# Autodesk Inventor assembly: ASY Disk Micro filter v2.0
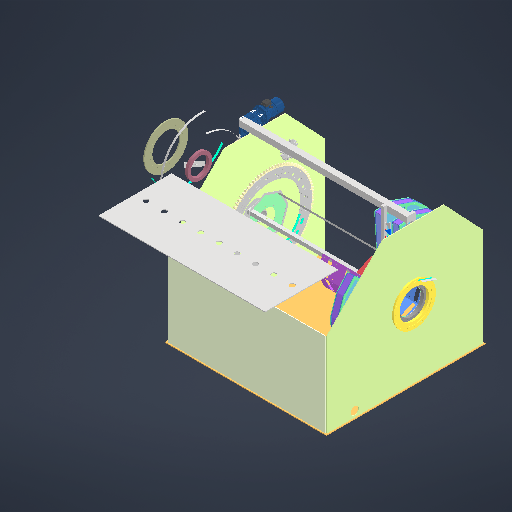
[picture p0: Inventor's stored thumbnail of the model, 512x512]
Saved by Autodesk Inventor 2026.2 (Build 302298010, 298A)
## iProperties
Created: 2023-08-31
Part Number: ASY Disk Micro filter v2.0
Document SubType Name: Assembly
Designer: admin
Stock Number: Дисковый_Фильтр
Author: admin
## Documents named in this file (38)
- C:\Users\admin\Documents\Inventor\DMF-Disk-Micro-Filter\ASY 000 ДМФ Disk Micro filter v2.0.iam
- C:\Users\admin\Documents\Inventor\DMF-Disk-Micro-Filter\Left wall v2.0.ipt
- C:\Users\admin\Documents\Inventor\DMF-Disk-Micro-Filter\Wall right v2.0.ipt
- C:\Users\admin\Documents\Inventor\DMF-Disk-Micro-Filter\DF1.03 Wall bottom v2.0.ipt
- C:\Users\admin\Documents\Inventor\DMF-Disk-Micro-Filter\DF1.04 Wall face v2.0.ipt
- C:\Users\admin\Documents\Inventor\DMF-Disk-Micro-Filter\ДМФ 021 кольцо прижимное нос v2.0.ipt
- C:\Users\admin\Documents\Inventor\DMF-Disk-Micro-Filter\ДМФ 000 размеры v2.0.ipt
- C:\Users\admin\Documents\Inventor\DMF-Disk-Micro-Filter\ДМФ 032 крышка Нос v2.0.ipt
- C:\Users\admin\Documents\Inventor\DMF-Disk-Micro-Filter\ДМФ 091 Постель НОС v2.0.ipt
- C:\Users\admin\Documents\Inventor\DMF-Disk-Micro-Filter\ДМФ 022 кольцо прижимное корма v2.0.ipt
- C:\Users\admin\Documents\Inventor\DMF-Disk-Micro-Filter\ДМФ 093 Постель КОРМА v2.0.ipt
- C:\Users\admin\Documents\Inventor\DMF-Disk-Micro-Filter\ДМФ 092 Коромысло КОРМА v2.0.ipt
- C:\Users\admin\Documents\Inventor\DMF-Disk-Micro-Filter\ДМФ 055 труба илоотвода v2.0.ipt
- C:\Users\admin\Documents\Inventor\DMF-Disk-Micro-Filter\ДМФ 033 держатель лотка v2.0.ipt
- C:\Users\admin\Documents\Inventor\DMF-Disk-Micro-Filter\ASY ДМФ лоток 050 илоотвод v2.0.iam
- C:\Users\admin\Documents\Inventor\DMF-Disk-Micro-Filter\ДМФ 092 Коромысло НОС v2.0.ipt
- C:\Users\admin\Documents\Inventor\DMF-Disk-Micro-Filter\ДМФ 066 Гребенка v2.0.ipt
- C:\Users\admin\Documents\Inventor\DMF-Disk-Micro-Filter\ДМФ 025 кольцо прижимное корма наружное v2.0.ipt
- C:\Users\admin\Documents\Inventor\DMF-Disk-Micro-Filter\ДМФ 067 крышка v2.0.ipt
- C:\Users\admin\Documents\Inventor\DMF-Disk-Micro-Filter\ДМФ 081 труба форсунки v2.0.ipt
- C:\Users\admin\Documents\Inventor\DMF-Disk-Micro-Filter\ASY Обрешетка лицевая стенка.iam
- C:\Users\admin\Documents\Inventor\DMF-Disk-Micro-Filter\ASY Консоль под двигатель вед. шестерни.iam
- C:\Users\admin\Documents\Inventor\DMF-Disk-Micro-Filter\Вал ведущей шестерни.ipt
- C:\Users\admin\Documents\Inventor\DMF-Disk-Micro-Filter\Корпусный подшипник D35.ipt
- C:\Users\admin\Documents\Inventor\DMF-Disk-Micro-Filter\Мотор-редуктор NMRV 090(80B5).ipt
- C:\Users\admin\Documents\Inventor\DMF-Disk-Micro-Filter\DMF pancake.ipt
- C:\Users\admin\Documents\Inventor\DMF-Disk-Micro-Filter\Нога для постели.ipt
- C:\Users\admin\Documents\Inventor\DMF-Disk-Micro-Filter\Нога для постели №2.ipt
- C:\Users\admin\Documents\Inventor\DMF-Disk-Micro-Filter\ДМФ 092 Постель НОС v2.0.ipt
- C:\Users\admin\Documents\Inventor\DMF-Disk-Micro-Filter\ДМФ 094 Постель НОС крепление v2.0.ipt
- C:\Users\admin\Documents\Inventor\DMF-Disk-Micro-Filter\DMF Hat 2.0.ipt
- C:\Users\admin\Documents\Inventor\DMF-Disk-Micro-Filter\DMF Flange exit 2.0.ipt
- C:\Users\admin\Documents\Inventor\DMF-Disk-Micro-Filter\Барабан v2.1\ASY ДМФ 0100 Барабан v2.1.iam
- C:\Users\admin\Documents\Inventor\DMF-Disk-Micro-Filter\Барабан v2.1\DMF flange small gear.ipt
- C:\Users\admin\Documents\Inventor\DMF-Disk-Micro-Filter\Барабан v2.1\DMF small gear.ipt
- C:\Users\admin\Documents\Inventor\DMF-Disk-Micro-Filter\DMF Support ring tail.ipt
- C:\Users\admin\Documents\Inventor\DMF-Disk-Micro-Filter\Промывка Алексенко\Промывка.iam
- C:\Users\admin\Documents\Inventor\DMF-Disk-Micro-Filter\DMF 082 коллектор болванка.ipt
## Components (38 placed, 38 different names)
1. ДМФ 000 размеры v2.0.ipt:1
2. Left wall v2.0.ipt:1 — Flush:4, Mate:1, Flush:6, Flush:7, Flush:9, Mate:4, Flush:26, Flush:27, Mate:25, Rigid:16, Rigid:27
3. Wall right v2.0.ipt:1 — Flush:23, Flush:24, Rigid:16, Rigid:32, Mate:32, Mate:33
4. DF1.03 Wall bottom v2.0.ipt:1 — Mate:1, Flush:6, Flush:7, Mate:3, Flush:11, Mate:24, Mate:30
5. DF1.04 Wall face v2.0.ipt:1 — Flush:9, Mate:3, Mate:4, Flush:10, Angle:1
6. ДМФ 021 кольцо прижимное нос v2.0.ipt:1
7. ДМФ 032 крышка Нос v2.0.ipt:1
8. ДМФ 091 Постель НОС v2.0.ipt:1
9. ДМФ 022 кольцо прижимное корма v2.0.ipt:1
10. ДМФ 093 Постель КОРМА v2.0.ipt:1
11. ДМФ 092 Коромысло КОРМА v2.0.ipt:1
12. ДМФ 055 труба илоотвода v2.0.ipt:1 — Rigid:26, Rigid:29
13. ДМФ 033 держатель лотка v2.0.ipt:1
14. ASY ДМФ лоток 050 илоотвод v2.0.iam:1 [sub-assembly]
15. ДМФ 092 Коромысло НОС v2.0.ipt:1
16. ДМФ 066 Гребенка v2.0.ipt:1 — Flush:22, Angle:1, Mate:24
17. ДМФ 025 кольцо прижимное корма наружное v2.0.ipt:1
18. ДМФ 067 крышка v2.0.ipt:1 — Flush:23, Flush:24
19. ASY Обрешетка лицевая стенка.iam:1 [sub-assembly] — Flush:26, Flush:27, Mate:25, Mate:26, Flush:28, Flush:30, Flush:34
20. ASY Консоль под двигатель вед. шестерни.iam:1 [sub-assembly] — Mate:26, Flush:28, Flush:30, Mate:28, Flush:31, Flush:32, Flush:33, Mate:31
21. Вал ведущей шестерни.ipt:1 — Rigid:30, Rigid:31
22. Корпусный подшипник D35.ipt:1 — Flush:33, Mate:31, Flush:34
23. Мотор-редуктор NMRV 090(80B5).ipt:1 — Mate:28, Flush:31, Rigid:30, Flush:32
24. DMF pancake.ipt:1 — Rigid:27, Rigid:28
25. Нога для постели.ipt:1
26. Нога для постели №2.ipt:1
27. ДМФ 092 Постель НОС v2.0.ipt:1
28. ДМФ 094 Постель НОС крепление v2.0.ipt:2
29. DMF Hat 2.0.ipt:1 — Rigid:28, Rigid:29
30. DMF Flange exit 2.0.ipt:1 — Rigid:26
31. ASY ДМФ 0100 Барабан v2.1:1 [sub-assembly] — Rotational:17, Rotational:18
32. flange small gear:1
33. DMF small gear:1 — Rigid:31
34. DMF Support ring tail:1 — Rigid:32, Rotational:17, Rotational:18
35. Промывка:1 [sub-assembly]
36. DMF 082 коллектор болванка:1 — Mate:32, Mate:33, Rigid:33, Rigid:34
37. ДМФ 081 труба форсунки v2.0:2 — Rigid:34
38. ДМФ 081 труба форсунки v2.0.ipt:1 — Rigid:33
## Relationships (42: Flush 17, Mate 12, WeldJoint 10, RevoluteJoint 2, Angle 1)
- Flush:4: Left wall v2.0.ipt:1
- Mate:1: Left wall v2.0.ipt:1 ↔ DF1.03 Wall bottom v2.0.ipt:1
- Flush:6 (15 mm): Left wall v2.0.ipt:1 ↔ DF1.03 Wall bottom v2.0.ipt:1
- Flush:7 (25 mm): Left wall v2.0.ipt:1 ↔ DF1.03 Wall bottom v2.0.ipt:1
- Flush:9: Left wall v2.0.ipt:1 ↔ DF1.04 Wall face v2.0.ipt:1
- Mate:3: DF1.03 Wall bottom v2.0.ipt:1 ↔ DF1.04 Wall face v2.0.ipt:1
- Mate:4: Left wall v2.0.ipt:1 ↔ DF1.04 Wall face v2.0.ipt:1
- Flush:10: DF1.04 Wall face v2.0.ipt:1
- Flush:11: DF1.03 Wall bottom v2.0.ipt:1
- [Mate]: ASY ДМФ лоток 050 илоотвод v2.0.iam:1
- Flush:22: ДМФ 066 Гребенка v2.0.ipt:1
- Angle:1 (180 deg): DF1.04 Wall face v2.0.ipt:1 ↔ ДМФ 066 Гребенка v2.0.ipt:1
- Mate:24: DF1.03 Wall bottom v2.0.ipt:1 ↔ ДМФ 066 Гребенка v2.0.ipt:1
- Flush:23: Wall right v2.0.ipt:1 ↔ ДМФ 067 крышка v2.0.ipt:1
- Flush:24 (-50 mm): Wall right v2.0.ipt:1 ↔ ДМФ 067 крышка v2.0.ipt:1
- Flush:26: Left wall v2.0.ipt:1 ↔ ASY Обрешетка лицевая стенка.iam:1
- Flush:27: Left wall v2.0.ipt:1 ↔ ASY Обрешетка лицевая стенка.iam:1
- Mate:25: Left wall v2.0.ipt:1 ↔ ASY Обрешетка лицевая стенка.iam:1
- Mate:26: ASY Обрешетка лицевая стенка.iam:1 ↔ ASY Консоль под двигатель вед. шестерни.iam:1
- Flush:28: ASY Обрешетка лицевая стенка.iam:1 ↔ ASY Консоль под двигатель вед. шестерни.iam:1
- Rigid:16 [WeldJoint] (2160 mm): Left wall v2.0.ipt:1 ↔ Wall right v2.0.ipt:1
- Flush:30: ASY Обрешетка лицевая стенка.iam:1 ↔ ASY Консоль под двигатель вед. шестерни.iam:1
- Mate:28: ASY Консоль под двигатель вед. шестерни.iam:1 ↔ Мотор-редуктор NMRV 090(80B5).ipt:1
- Flush:31: ASY Консоль под двигатель вед. шестерни.iam:1 ↔ Мотор-редуктор NMRV 090(80B5).ipt:1
- Mate:30: DF1.03 Wall bottom v2.0.ipt:1
- Rigid:26 [WeldJoint]: ДМФ 055 труба илоотвода v2.0.ipt:1 ↔ DMF Flange exit 2.0.ipt:1
- Rigid:27 [WeldJoint]: Left wall v2.0.ipt:1 ↔ DMF pancake.ipt:1
- Rigid:28 [WeldJoint]: DMF pancake.ipt:1 ↔ DMF Hat 2.0.ipt:1
- Rigid:29 [WeldJoint] (100 mm): ДМФ 055 труба илоотвода v2.0.ipt:1 ↔ DMF Hat 2.0.ipt:1
- Rigid:30 [WeldJoint]: Вал ведущей шестерни.ipt:1 ↔ Мотор-редуктор NMRV 090(80B5).ipt:1
- Flush:32 (47 mm): ASY Консоль под двигатель вед. шестерни.iam:1 ↔ Мотор-редуктор NMRV 090(80B5).ipt:1
- Rigid:31 [WeldJoint]: Вал ведущей шестерни.ipt:1 ↔ DMF small gear:1
- Flush:33 (66.5 mm): ASY Консоль под двигатель вед. шестерни.iam:1 ↔ Корпусный подшипник D35.ipt:1
- Mate:31 (55.4 mm): ASY Консоль под двигатель вед. шестерни.iam:1 ↔ Корпусный подшипник D35.ipt:1
- Flush:34: ASY Обрешетка лицевая стенка.iam:1 ↔ Корпусный подшипник D35.ipt:1
- Rigid:32 [WeldJoint]: Wall right v2.0.ipt:1 ↔ DMF Support ring tail:1
- Rotational:17 [RevoluteJoint]: ASY ДМФ 0100 Барабан v2.1:1 ↔ DMF Support ring tail:1
- Rotational:18 [RevoluteJoint]: ASY ДМФ 0100 Барабан v2.1:1 ↔ DMF Support ring tail:1
- Mate:32: Wall right v2.0.ipt:1 ↔ DMF 082 коллектор болванка:1
- Mate:33 (20 mm): Wall right v2.0.ipt:1 ↔ DMF 082 коллектор болванка:1
- Rigid:33 [WeldJoint]: DMF 082 коллектор болванка:1 ↔ ДМФ 081 труба форсунки v2.0.ipt:1
- Rigid:34 [WeldJoint] (-280 mm): DMF 082 коллектор болванка:1 ↔ ДМФ 081 труба форсунки v2.0:2
